# Autodesk Inventor assembly: Zahnstange
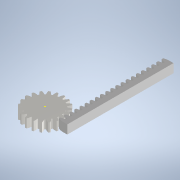
[picture p0: Inventor's stored thumbnail of the model, 180x180]
Saved by Autodesk Inventor 2021 (Build 250183000, 183)
## iProperties
Created: 2021-01-13
Part Number: Zahnstange
Document SubType Name: Assembly
Designer: LETPJG
Author: LETPJG
## Documents named in this file (3)
- C:\Users\LETPJG\Documents\Inventor\zahnstange\Zahnstange.iam
- C:\Users\LETPJG\Documents\Inventor\zahnstange\Zahnstange\Konstruktions-Assistent\Stirnräder11.iam
- C:\Users\LETPJG\Documents\Inventor\zahnstange\Zahnstange.ipt
## Components (2 placed, 2 different names)
1. Stirnräder:1 [sub-assembly] — Fluchtend:1, Passend:1, Fluchtend:2, Fluchtend:3, Fluchtend:5, Drehung/Translation:1, Winkel:1
2. Zahnstange:1 — Fluchtend:2, Fluchtend:3, Fluchtend:4, Fluchtend:5, Drehung/Translation:1
## Relationships (8: Flush 5, Mate 1, RelateRotateTranslate 1, Angle 1)
- Fluchtend:1 [Flush]: Stirnräder:1
- Passend:1 [Mate]: Stirnräder:1
- Fluchtend:2 [Flush]: Stirnräder:1 ↔ Zahnstange:1
- Fluchtend:3 [Flush]: Stirnräder:1 ↔ Zahnstange:1
- Fluchtend:4 [Flush] (-15 mm): Zahnstange:1
- Fluchtend:5 [Flush] (-2.39 mm): Stirnräder:1 ↔ Zahnstange:1
- Drehung/Translation:1 [RelateRotateTranslate] (62.8319 mm): Stirnräder:1 ↔ Zahnstange:1
- Winkel:1 [Angle] (0 deg): Stirnräder:1
